# Autodesk Inventor assembly: 9P Sprocket
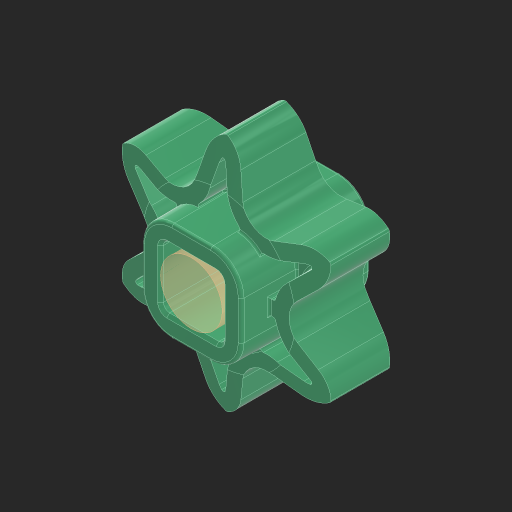
[picture p0: Inventor's stored thumbnail of the model, 512x512]
Saved by Autodesk Inventor 2023 (Build 270158000, 158)
## iProperties
Created: 2022-08-02
Part Number: 9P Sprocket
Document SubType Name: Assembly
Designer: ylu12
Author: ylu12
## Documents named in this file (23)
- C:\Users\ylu12\Documents\GitHub\VEX-CAD-Inventor\Motion\Sprockets\9P Sprocket.iam
- C:\Users\ylu12\Documents\GitHub\VEX-CAD-Inventor\Motion\HS Shaft Adapter Circle.ipt
- C:\Users\ylu12\Documents\GitHub\VEX-CAD-Inventor\Motion\HS Shaft Adapter Square.ipt
- C:\Users\ylu12\Documents\GitHub\VEX-CAD-Inventor\Motion\Sprockets\Reference Files\9P 6T Sprocket, No Insert.ipt
- C:\Users\ylu12\Documents\GitHub\VEX-CAD-Inventor\Motion\Sprockets\Reference Files\9P 12T Sprocket, No Insert.ipt
- C:\Users\ylu12\Documents\GitHub\VEX-CAD-Inventor\Motion\Sprockets\Reference Files\9P 18T Sprocket, No Insert.ipt
- C:\Users\ylu12\Documents\GitHub\VEX-CAD-Inventor\Motion\Sprockets\Reference Files\9P 24T Sprocket, No Insert.ipt
- C:\Users\ylu12\Documents\GitHub\VEX-CAD-Inventor\Motion\Sprockets\Reference Files\9P 30T Sprocket, No Insert.ipt
- 9P 12T Sprocket, Circle.iam
- 9P 12T Sprocket, No Insert.iam
- 9P 12T Sprocket, Square.iam
- 9P 18T Sprocket, Circle.iam
- 9P 18T Sprocket, No Insert.iam
- 9P 18T Sprocket, Square.iam
- 9P 24T Sprocket, Circle.iam
- 9P 24T Sprocket, No Insert.iam
- 9P 24T Sprocket, Square.iam
- 9P 30T Sprocket, Circle.iam
- 9P 30T Sprocket, No Insert.iam
- 9P 30T Sprocket, Square.iam
- 9P 6T Sprocket, Circle.iam
- 9P 6T Sprocket, No Insert.iam
- 9P 6T Sprocket, Square.iam
## Components (7 placed, 7 different names)
1. Circle — Mate:1, Mate:2, Flush:1
2. Square — Mate:3, Mate:4, Flush:2
3. 6T — Mate:5, Mate:6, Flush:3
4. 12T — Mate:7, Mate:8, Flush:4
5. 18T — Flush:5, Mate:9, Mate:10
6. 24T — Flush:6, Mate:11, Mate:12
7. 30T — Mate:14, Mate:15, Mate:16
## Relationships (21: Mate 15, Flush 6)
- Mate:1: Circle
- Mate:2: Circle
- Mate:3: Square
- Mate:4: Square
- Flush:1 (6.35 mm): Circle
- Flush:2 (6.35 mm): Square
- Mate:5: 6T
- Mate:6: 6T
- Flush:3: 6T
- Mate:7: 12T
- Mate:8: 12T
- Flush:4: 12T
- Flush:5: 18T
- Flush:6: 24T
- Mate:9: 18T
- Mate:10: 18T
- Mate:11: 24T
- Mate:12: 24T
- Mate:14: 30T
- Mate:15: 30T
- Mate:16: 30T
